# Autodesk Inventor assembly: A2017_T4_11
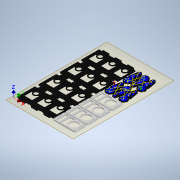
[picture p0: Inventor's stored thumbnail of the model, 180x180]
Saved by Autodesk Inventor 2020 (Build 240168000, 168)
## iProperties
Created: 2021-08-27
Part Number: A2017_T4_11
Document SubType Name: Assembly
Designer: Masato
Author: Masato
## Documents named in this file (5)
- D:\GitHub\inventor\SUSTAINA-OP\Cam\A2017_T4_11.iam
- D:\GitHub\inventor\SUSTAINA-OP\Cam\DisposableBoard.ipt
- D:\GitHub\inventor\SUSTAINA-OP\UpperBody\Trunk\Trunk_neck_frame.ipt
- D:\GitHub\inventor\SUSTAINA-OP\UpperBody\Trunk\Trunk_servo_bottom_frame.ipt
- D:\GitHub\inventor\SUSTAINA-OP\LowerBody\Ankle\Ankle_side_pitch_frame.ipt
## Components (29 placed, 4 different names)
1. DisposableBoard:1 — メイト:2, メイト:1, フラッシュ:1, フラッシュ:2, メイト:8, フラッシュ:5, フラッシュ:6, メイト:10, メイト:12, メイト:13, メイト:14
2. Ankle_side_pitch_frame:1 — メイト:12, 正接:1, 正接:2, 角度:1, メイト:15
3. Ankle_side_pitch_frame:2 — メイト:13, 正接:3, メイト:15, メイト:16
4. Ankle_side_pitch_frame:3 — メイト:14, 正接:4, メイト:16
5. Ankle_side_pitch_frame:4
6. Ankle_side_pitch_frame:5
7. Ankle_side_pitch_frame:6
8. Trunk_neck_frame:2 — メイト:10, フラッシュ:7, メイト:11
9. Trunk_neck_frame:3
10. Trunk_neck_frame:4
11. Trunk_neck_frame:5 — 正接:1, 正接:3, 正接:4
12. Trunk_servo_bottom_frame:1 — メイト:8, フラッシュ:5, フラッシュ:6, フラッシュ:7
13. Trunk_servo_bottom_frame:2
14. Trunk_servo_bottom_frame:3 — メイト:11
15. Trunk_servo_bottom_frame:4
16. Trunk_servo_bottom_frame:5
17. Trunk_servo_bottom_frame:6
18. Trunk_servo_bottom_frame:7
19. Trunk_servo_bottom_frame:8
20. Trunk_servo_bottom_frame:9
21. Trunk_servo_bottom_frame:10
22. Trunk_servo_bottom_frame:11
23. Trunk_servo_bottom_frame:12 — 正接:2
24. Trunk_servo_bottom_frame:13
25. Trunk_servo_bottom_frame:14
26. Trunk_servo_bottom_frame:15
27. Trunk_servo_bottom_frame:16
28. Trunk_servo_bottom_frame:17
29. Trunk_servo_bottom_frame:18
## Component patterns: (2 elements), (3 elements), (2 elements, first: Ankle_side_pitch_frame:1 + Ankle_side_pitch_frame:2 + Ankle_side_pitch_frame:3), (2 elements, first: Trunk_neck_frame:2), コンポーネント パターン 3:2 (2 elements), (2 elements), コンポーネント パターン 4:2 (2 elements), コンポーネント パターン 4:3 (2 elements), (3 elements, first: Trunk_servo_bottom_frame:1), コンポーネント パターン 2:2 (3 elements), コンポーネント パターン 2:3 (3 elements), コンポーネント パターン 2:4 (3 elements), コンポーネント パターン 2:5 (3 elements), コンポーネント パターン 2:6 (3 elements)
## Relationships (20: Mate 10, Flush 5, Tangent 4, Angle 1)
- メイト:2 [Mate]: DisposableBoard:1
- メイト:1 [Mate]: DisposableBoard:1
- フラッシュ:1 [Flush]: DisposableBoard:1
- フラッシュ:2 [Flush]: DisposableBoard:1
- メイト:8 [Mate]: DisposableBoard:1 ↔ Trunk_servo_bottom_frame:1
- フラッシュ:5 [Flush] (5 mm): DisposableBoard:1 ↔ Trunk_servo_bottom_frame:1
- フラッシュ:6 [Flush] (2 mm): DisposableBoard:1 ↔ Trunk_servo_bottom_frame:1
- メイト:10 [Mate]: DisposableBoard:1 ↔ Trunk_neck_frame:2
- フラッシュ:7 [Flush]: Trunk_neck_frame:2 ↔ Trunk_servo_bottom_frame:1
- メイト:11 [Mate] (2.5 mm): Trunk_neck_frame:2 ↔ Trunk_servo_bottom_frame:3
- メイト:12 [Mate]: DisposableBoard:1 ↔ Ankle_side_pitch_frame:1
- メイト:13 [Mate]: DisposableBoard:1 ↔ Ankle_side_pitch_frame:2
- メイト:14 [Mate]: DisposableBoard:1 ↔ Ankle_side_pitch_frame:3
- 正接:1 [Tangent] (2.5 mm): Ankle_side_pitch_frame:1 ↔ Trunk_neck_frame:5
- 正接:2 [Tangent] (2.5 mm): Ankle_side_pitch_frame:1 ↔ Trunk_servo_bottom_frame:12
- 正接:3 [Tangent] (2.5 mm): Ankle_side_pitch_frame:2 ↔ Trunk_neck_frame:5
- 正接:4 [Tangent] (2.5 mm): Ankle_side_pitch_frame:3 ↔ Trunk_neck_frame:5
- 角度:1 [Angle] (90 deg): Ankle_side_pitch_frame:1
- メイト:15 [Mate] (2.5 mm): Ankle_side_pitch_frame:1 ↔ Ankle_side_pitch_frame:2
- メイト:16 [Mate] (2.5 mm): Ankle_side_pitch_frame:2 ↔ Ankle_side_pitch_frame:3
